# Autodesk Inventor assembly: 前脚ギアトレイン5
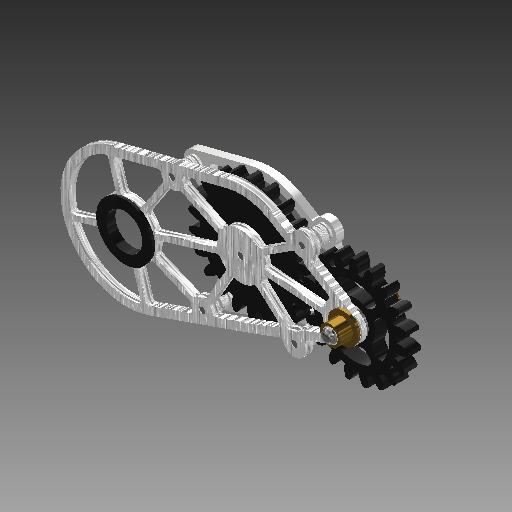
[picture p0: Inventor's stored thumbnail of the model, 512x512]
Saved by Autodesk Inventor 2020 (Build 240168000, 168)
## iProperties
Created: 2019-09-03
Part Number: 前脚ギアトレイン5
Document SubType Name: Assembly
Designer: 雪村
Mass: 56.2164 g
Surface Area: 264.788 cm^2
Volume: 20.7039 cm^3
Density: 2.71525 g/cm^3
Author: 雪村
## Documents named in this file (11)
- C:\Users\white\Documents\SRDC\SRDC\Inventor_2017\2018年機体\2020年4年機体\前脚ギアトレイン5.iam
- C:\Users\white\Documents\SRDC\SRDC\Inventor_2017\2018年機体\2020年4年機体\前脚ギアトレイン5.1.ipt
- C:\Users\white\Documents\SRDC\SRDC\Inventor_2017\2018年機体\2020年4年機体\前脚ギアトレイン5.2.ipt
- C:\Users\white\Documents\SRDC\SRDC\Inventor_2017\2018年機体\2020年4年機体\歯車m2.z22.ipt
- C:\Users\white\Documents\SRDC\SRDC\Inventor_2017\2018年機体\2020年4年機体\歯車m2.z19.ipt
- C:\Users\white\Documents\SRDC\SRDC\Inventor_2017\2018年機体\パーツ\ベアリングフランジ付き0610.3t.ipt
- C:\Users\white\Documents\SRDC\SRDC\Inventor_2017\2018年機体\パーツ\スペーサーm3,7.ipt
- C:\Users\white\Documents\SRDC\SRDC\Inventor_2017\2018年機体\パーツ\オイレスフランジ付き14162202.5.ipt
- C:\Users\white\Documents\SRDC\SRDC\Inventor_2017\2018年機体\パーツ\オイレスフランジ付き06080512,1t ドライメット.ipt
- C:\Users\white\Documents\SRDC\SRDC\Inventor_2017\2018年機体\パーツ\スペーサーm3,6.ipt
- C:\Users\white\Documents\SRDC\SRDC\Inventor_2017\2018年機体\パーツ\ネジ鍋m3,12.ipt
## Components (26 placed, 10 different names)
1. 前脚ギアトレイン5.1:1 — 挿入:5, 挿入:6, 挿入:8, 挿入:9, 挿入:10, 挿入:11, 挿入:12, 挿入:13, 挿入:14, 挿入:16, 挿入:18
2. 前脚ギアトレイン5.2:1 — メイト:1, 挿入:7, 挿入:15, 挿入:17, 挿入:21, 挿入:22, 挿入:23, 挿入:24, 挿入:25
3. 歯車m2.z22:1 — 挿入:3, 挿入:4
4. 歯車m2.z19:1 — 挿入:1, 挿入:2
5. ベアリングフランジ付き0610.3t:1 — 挿入:1, メイト:1
6. ベアリングフランジ付き0610.3t:2 — 挿入:2, 挿入:5
7. ベアリングフランジ付き0610.3t:3 — 挿入:3, 挿入:7
8. ベアリングフランジ付き0610.3t:4 — 挿入:4, 挿入:6
9. スペーサーm3,7:1 — 挿入:9
10. スペーサーm3,7:2 — 挿入:8
11. スペーサーm3,7:3 — 挿入:10
12. スペーサーm3,7:4 — 挿入:13
13. スペーサーm3,7:5 — 挿入:11
14. スペーサーm3,7:6 — 挿入:12
15. オイレスフランジ付き14162202.5:1 — 挿入:14
16. オイレスフランジ付き06080512,1t ドライメット:1 — 挿入:15, 挿入:19
17. オイレスフランジ付き06080512,1t ドライメット:2 — 挿入:16
18. スペーサーm3,6:1 — 挿入:17
19. スペーサーm3,6:2 — 挿入:18, 挿入:20
20. ネジ鍋m3,12:1 — 挿入:19
21. ネジ鍋m3,12:2 — 挿入:20
22. ネジ鍋m3,12:3 — 挿入:25
23. ネジ鍋m3,12:4 — 挿入:22
24. ネジ鍋m3,12:5 — 挿入:24
25. ネジ鍋m3,12:6 — 挿入:21
26. ネジ鍋m3,12:7 — 挿入:23
## Relationships (26: Insert 25, Mate 1)
- 挿入:1 [Insert]: 歯車m2.z19:1 ↔ ベアリングフランジ付き0610.3t:1
- 挿入:2 [Insert]: 歯車m2.z19:1 ↔ ベアリングフランジ付き0610.3t:2
- 挿入:3 [Insert]: 歯車m2.z22:1 ↔ ベアリングフランジ付き0610.3t:3
- 挿入:4 [Insert]: 歯車m2.z22:1 ↔ ベアリングフランジ付き0610.3t:4
- 挿入:5 [Insert]: 前脚ギアトレイン5.1:1 ↔ ベアリングフランジ付き0610.3t:2
- 挿入:6 [Insert]: 前脚ギアトレイン5.1:1 ↔ ベアリングフランジ付き0610.3t:4
- メイト:1 [Mate]: 前脚ギアトレイン5.2:1 ↔ ベアリングフランジ付き0610.3t:1
- 挿入:7 [Insert]: 前脚ギアトレイン5.2:1 ↔ ベアリングフランジ付き0610.3t:3
- 挿入:8 [Insert]: 前脚ギアトレイン5.1:1 ↔ スペーサーm3,7:2
- 挿入:9 [Insert]: 前脚ギアトレイン5.1:1 ↔ スペーサーm3,7:1
- 挿入:10 [Insert]: 前脚ギアトレイン5.1:1 ↔ スペーサーm3,7:3
- 挿入:11 [Insert]: 前脚ギアトレイン5.1:1 ↔ スペーサーm3,7:5
- 挿入:12 [Insert]: 前脚ギアトレイン5.1:1 ↔ スペーサーm3,7:6
- 挿入:13 [Insert]: 前脚ギアトレイン5.1:1 ↔ スペーサーm3,7:4
- 挿入:14 [Insert]: 前脚ギアトレイン5.1:1 ↔ オイレスフランジ付き14162202.5:1
- 挿入:15 [Insert]: 前脚ギアトレイン5.2:1 ↔ オイレスフランジ付き06080512,1t ドライメット:1
- 挿入:16 [Insert]: 前脚ギアトレイン5.1:1 ↔ オイレスフランジ付き06080512,1t ドライメット:2
- 挿入:17 [Insert]: 前脚ギアトレイン5.2:1 ↔ スペーサーm3,6:1
- 挿入:18 [Insert]: 前脚ギアトレイン5.1:1 ↔ スペーサーm3,6:2
- 挿入:19 [Insert]: オイレスフランジ付き06080512,1t ドライメット:1 ↔ ネジ鍋m3,12:1
- 挿入:20 [Insert]: スペーサーm3,6:2 ↔ ネジ鍋m3,12:2
- 挿入:21 [Insert]: 前脚ギアトレイン5.2:1 ↔ ネジ鍋m3,12:6
- 挿入:22 [Insert]: 前脚ギアトレイン5.2:1 ↔ ネジ鍋m3,12:4
- 挿入:23 [Insert]: 前脚ギアトレイン5.2:1 ↔ ネジ鍋m3,12:7
- 挿入:24 [Insert]: 前脚ギアトレイン5.2:1 ↔ ネジ鍋m3,12:5
- 挿入:25 [Insert]: 前脚ギアトレイン5.2:1 ↔ ネジ鍋m3,12:3
